# Autodesk Inventor assembly: manipulator
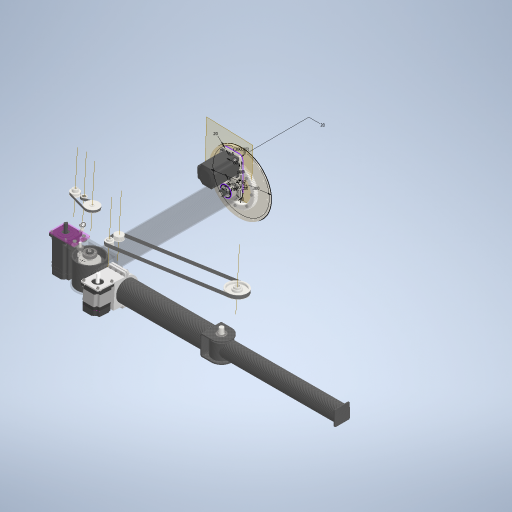
[picture p0: Inventor's stored thumbnail of the model, 512x512]
Saved by Autodesk Inventor 2023 (Build 270158000, 158)
## iProperties
Created: 2023-03-28
Part Number: manipulator
Document SubType Name: Assembly
Designer: krzys
Mass: 18520.6 g
Surface Area: 24173.7 cm^2
Volume: 7260.75 cm^3
Author: krzys
## Documents named in this file (36)
- C:\Users\krzys\Documents\GitHub\Manipulator-Inventor\Manipulator.iam
- C:\Users\krzys\Documents\GitHub\Manipulator-Inventor\podstawa.ipt
- C:\Users\krzys\Documents\GitHub\Manipulator-Inventor\podstwa_obrotowa.ipt
- C:\Users\krzys\Documents\GitHub\Manipulator-Inventor\CS-M23480_3D.ipt
- C:\Users\krzys\Documents\GitHub\Manipulator-Inventor\czlon 1 i 2.iam
- C:\Users\krzys\Documents\GitHub\Manipulator-Inventor\Manipulator\Design Accelerator\Łożysko6.iam
- C:\Users\krzys\Documents\GitHub\Manipulator-Inventor\Wał2.ipt
- C:\Users\krzys\Documents\GitHub\Manipulator-Inventor\Manipulator\Design Accelerator\Przekładnie walcowe1.iam
- C:\Users\krzys\Documents\GitHub\Manipulator-Inventor\czlon 3.ipt
- C:\Users\krzys\Documents\GitHub\Manipulator-Inventor\mocowanie silnika.ipt
- C:\Users\krzys\Documents\GitHub\Manipulator-Inventor\silniki\CS-M23485B_3D.ipt
- C:\Users\krzys\Documents\GitHub\Manipulator-Inventor\Manipulator\Design Accelerator\Przekładnie pasowe synchroniczne1.iam
- C:\Users\krzys\Documents\GitHub\Manipulator-Inventor\mocowanie_silnika_członu_3.ipt
- C:\Users\krzys\Documents\GitHub\Manipulator-Inventor\Manipulator\Design Accelerator\Przekładnie pasowe synchroniczne2.iam
- C:\Users\krzys\Documents\GitHub\Manipulator-Inventor\silniki\CS-M23445WP\CS-M23445WP_3D.iam
- C:\Users\krzys\Documents\GitHub\Manipulator-Inventor\Manipulator\Design Accelerator\Łożysko5.iam
- C:\Users\krzys\Documents\GitHub\Manipulator-Inventor\podkladka.ipt
- C:\Users\krzys\Documents\GitHub\Manipulator-Inventor\podkladka_os2.ipt
- C:\Users\krzys\Documents\Inventor\Content Center Files\R2023\pl-PL\ISO 4034(1)\ISO 4034 - M16DIN EN.ipt
- C:\Users\krzys\Documents\Inventor\Content Center Files\R2023\pl-PL\DIN 933\DIN 933 - M6  x 30.ipt
- C:\Users\krzys\Documents\Inventor\Content Center Files\R2023\pl-PL\ISO 7089\ISO 7089 - 6 - 140 HV(1).ipt
- C:\Users\krzys\Documents\Inventor\Content Center Files\R2023\pl-PL\DIN 934\DIN 934 - M6 x 1.ipt
- C:\Users\krzys\Documents\Inventor\Content Center Files\R2023\pl-PL\DIN 912\DIN 912 - M6 x 1 x 25 x 22,5.ipt
- C:\Users\krzys\Documents\Inventor\Content Center Files\R2023\pl-PL\DIN 125-1  A\DIN 125 - A 6,4.ipt
- C:\Users\krzys\Documents\Inventor\Content Center Files\R2023\pl-PL\DIN 912\DIN 912 - M6 x 1 x 20 x 17,5.ipt
- C:\Users\krzys\Documents\Inventor\Content Center Files\R2023\pl-PL\DIN 912\DIN 912 - M6 x 1 x 30 x 27,5.ipt
- C:\Users\krzys\Documents\Inventor\Content Center Files\R2023\pl-PL\DIN 933\DIN 933 - M8  x 22.ipt
- C:\Users\krzys\Documents\Inventor\Content Center Files\R2023\pl-PL\DIN 9021\DIN 9021 - 8,4.ipt
- C:\Users\krzys\Documents\Inventor\Content Center Files\R2023\pl-PL\DIN 934\DIN 934 - M8 x 1,25.ipt
- C:\Users\krzys\Documents\Inventor\Content Center Files\R2023\pl-PL\DIN 6921\DIN 6921 - M6 x 16 - A.ipt
- C:\Users\krzys\Documents\GitHub\Manipulator-Inventor\Manipulator\Design Accelerator\Łożysko7.iam
- C:\Users\krzys\Documents\GitHub\Manipulator-Inventor\Wał4.ipt
- C:\Users\krzys\Documents\Inventor\Content Center Files\R2023\pl-PL\DIN 127 - W\DIN 127 - A 6.ipt
- C:\Users\krzys\Documents\Inventor\Content Center Files\R2023\pl-PL\DIN 6921\DIN 6921 - M6 x 30 - A.ipt
- C:\Users\krzys\Documents\GitHub\Manipulator-Inventor\Manipulator\Design Accelerator\Przekładnie walcowe2.iam
- C:\Users\krzys\Documents\Inventor\Content Center Files\R2023\pl-PL\DIN 933\DIN 933 - M6  x 28.ipt
## Components (101 placed, 30 different names)
1. podstawa:1 — Wstawiające:6, Zestawiające:9, Zestawiające:80, Równoległe:7, Równoległe:8, Równoległe:9
2. podstwa_obrotowa:1 — Wstawiające:11, Wstawiające:8, Wstawiające:9, Wstawiające:25, Wstawiające:26, Wstawiające:27, Wstawiające:28, Zestawiające:52, Wstawiające:33, Wstawiające:34, Wstawiające:35, Wstawiające:36, Wstawiające:48
3. CS-M23480_3D:1 — Wstawiające:9, Wstawiające:29, Wstawiające:30, Wstawiające:31, Wstawiające:32, Zestawiające:79, Równoległe:5
4. czlon 1 i 2:1 [sub-assembly] — Wstawiające:11, Wstawiające:1, Zestawiające:6, Wstawiające:4, Wstawiające:12, Wstawiające:13, Wstawiające:14, Zestawiające:60, Zestawiające:62, Zestawiające:69, przesuwne:2
5. Łożysko:3 [sub-assembly] — Wstawiające:1, Zestawiające:72, Równoległe:4, Kątowe:1
6. Wał:1 — Zestawiające:5, Równoległe:2, Równoległe:3, Zestawiające:72, Równoległe:4, Kątowe:1
7. Przekładnie walcowe:1 [sub-assembly] — Zestawiające:5, Równoległe:2, Zestawiające:6, Równoległe:3
8. czlon 3:1 — Wstawiające:12
9. mocowanie silnika:1 — Wstawiające:38, Wstawiające:39, Wstawiające:40, Wstawiające:41, przesuwne:2
10. CS-M23485B_3D:1 — Wstawiające:40, Wstawiające:41, Wstawiające:42, Wstawiające:43, Wstawiające:44, Wstawiające:45
11. Przekładnie pasowe synchroniczne:1 [sub-assembly] — Wstawiające:46, Zestawiające:73
12. mocowanie_silnika_członu_3:1 — Wstawiające:4, Zestawiające:11, Zestawiające:12, Zestawiające:13, Zestawiające:14, Zestawiające:15, Zestawiające:16, Zestawiające:17, Zestawiające:18, Zestawiające:19, Zestawiające:20, Zestawiające:21, Zestawiające:22, Zestawiające:23, Zestawiające:24, Zestawiające:25, Zestawiające:26, Zestawiające:27, Zestawiające:28, Zestawiające:29, Zestawiające:30, Zestawiające:31, Zestawiające:32, Zestawiające:33, Zestawiające:34, Wstawiające:21, Wstawiające:22, Wstawiające:23, Wstawiające:24, Wstawiające:65
13. Przekładnie pasowe synchroniczne:2 [sub-assembly]
14. CS-M23445WP_3D:1 [sub-assembly] — Wstawiające:65, Wstawiające:66, Wstawiające:67, Wstawiające:68, Wstawiające:69
15. Łożysko:4 [sub-assembly] — Wstawiające:6, Wstawiające:48
16. Łożysko:5 [sub-assembly] — Wstawiające:8, Wstawiające:10
17. podkladka:1 — Wstawiające:10, Zestawiające:10
18. podkladka_os2:1 — Wstawiające:13, Zestawiające:8, Zestawiające:67, Zestawiające:68
19. podkladka_os2:2 — Wstawiające:14, Zestawiające:70
20. DIN EN 24034 M16:1 — Zestawiające:9, Zestawiające:10
21. DIN 933 - zastąpiona przez DIN EN 24017 M6  x 30:1 — Zestawiające:11, Zestawiające:12
22. ISO 7089 6:1 — Zestawiające:13, Zestawiające:14, Wstawiające:15
23. DIN 934 - zastąpiona przez DIN EN 24032/28673/28674 M6:1 — Wstawiające:15
24. DIN 933 - zastąpiona przez DIN EN 24017 M6  x 30:2 — Zestawiające:15, Zestawiające:16
25. ISO 7089 6:2 — Zestawiające:17, Zestawiające:18, Wstawiające:16
26. DIN 934 - zastąpiona przez DIN EN 24032/28673/28674 M6:2 — Wstawiające:16
27. DIN 933 - zastąpiona przez DIN EN 24017 M6  x 30:3 — Zestawiające:19, Zestawiające:20
28. ISO 7089 6:3 — Zestawiające:21, Zestawiające:22, Wstawiające:17
29. DIN 934 - zastąpiona przez DIN EN 24032/28673/28674 M6:3 — Wstawiające:17
30. DIN 933 - zastąpiona przez DIN EN 24017 M6  x 30:4 — Zestawiające:23, Zestawiające:24
31. ISO 7089 6:4 — Zestawiające:25, Zestawiające:26, Wstawiające:18
32. DIN 934 - zastąpiona przez DIN EN 24032/28673/28674 M6:4 — Wstawiające:18
33. DIN 933 - zastąpiona przez DIN EN 24017 M6  x 30:5 — Zestawiające:27, Zestawiające:28
34. ISO 7089 6:5 — Zestawiające:29, Zestawiające:30, Wstawiające:19
35. DIN 934 - zastąpiona przez DIN EN 24032/28673/28674 M6:5 — Wstawiające:19
36. DIN 933 - zastąpiona przez DIN EN 24017 M6  x 30:6 — Zestawiające:31, Zestawiające:32
37. ISO 7089 6:6 — Zestawiające:33, Zestawiające:34, Wstawiające:20
38. DIN 934 - zastąpiona przez DIN EN 24032/28673/28674 M6:6 — Wstawiające:20
39. DIN 125-1 A A 6,4:1 — Wstawiające:21, Wstawiające:73
40. DIN 125-1 A A 6,4:2 — Wstawiające:22, Wstawiające:70
41. DIN 125-1 A A 6,4:3 — Wstawiające:23, Wstawiające:72
42. DIN 125-1 A A 6,4:4 — Wstawiające:24, Wstawiające:71
43. DIN 912 - zastąpiona przez DIN EN ISO 4762 M6 x 20:1 — Wstawiające:25
44. DIN 912 - zastąpiona przez DIN EN ISO 4762 M6 x 20:2 — Wstawiające:26
45. DIN 912 - zastąpiona przez DIN EN ISO 4762 M6 x 20:3 — Wstawiające:27
46. DIN 912 - zastąpiona przez DIN EN ISO 4762 M6 x 20:4 — Wstawiające:28
47. DIN 912 - zastąpiona przez DIN EN ISO 4762 M6 x 30:1 — Wstawiające:29, Zestawiające:51, Zestawiające:53
48. DIN 912 - zastąpiona przez DIN EN ISO 4762 M6 x 30:2 — Wstawiające:30, Zestawiające:55
49. DIN 912 - zastąpiona przez DIN EN ISO 4762 M6 x 30:3 — Wstawiające:31, Zestawiające:57
50. DIN 912 - zastąpiona przez DIN EN ISO 4762 M6 x 30:4 — Wstawiające:32
51. DIN 125-1 A A 6,4:5 — Zestawiające:51, Zestawiające:52, Zestawiające:54
52. DIN 125-1 A A 6,4:6 — Wstawiające:33, Zestawiające:56
53. DIN 125-1 A A 6,4:7 — Wstawiające:34, Wstawiające:37
54. DIN 125-1 A A 6,4:8 — Wstawiające:35
55. DIN 125-1 A A 6,4:9 — Wstawiające:36, Zestawiające:58
56. DIN 934 - zastąpiona przez DIN EN 24032/28673/28674 M6:11 — Zestawiające:53, Zestawiające:54
57. DIN 934 - zastąpiona przez DIN EN 24032/28673/28674 M6:12 — Zestawiające:55, Zestawiające:56
58. DIN 934 - zastąpiona przez DIN EN 24032/28673/28674 M6:13 — Wstawiające:37
59. DIN 934 - zastąpiona przez DIN EN 24032/28673/28674 M6:14 — Zestawiające:57, Zestawiające:58
60. DIN 933 - zastąpiona przez DIN EN 24017 M8  x 22:1 — Wstawiające:38, Zestawiające:59, Zestawiające:63
61. DIN 933 - zastąpiona przez DIN EN 24017 M8  x 22:2 — Wstawiające:39, Zestawiające:61, Zestawiające:65
62. DIN 9021 8,4:1 — Zestawiające:59, Zestawiające:60, Zestawiające:64
63. DIN 9021 8,4:2 — Zestawiające:61, Zestawiające:62, Zestawiające:66
64. DIN 934 - zastąpiona przez DIN EN 24032/28673/28674 M8:1 — Zestawiające:63, Zestawiające:64
65. DIN 934 - zastąpiona przez DIN EN 24032/28673/28674 M8:2 — Zestawiające:65, Zestawiające:66
66. DIN 912 - zastąpiona przez DIN EN ISO 4762 M6 x 20:5 — Wstawiające:42
67. DIN 912 - zastąpiona przez DIN EN ISO 4762 M6 x 20:6 — Wstawiające:43
68. DIN 912 - zastąpiona przez DIN EN ISO 4762 M6 x 20:7 — Wstawiające:44
69. DIN 912 - zastąpiona przez DIN EN ISO 4762 M6 x 20:8 — Wstawiające:45
70. DIN 6921 M6 x 16:1 — Zestawiające:67, Zestawiające:68
71. DIN 6921 M6 x 16:2 — Zestawiające:69, Zestawiające:70
72. Łożysko:6 [sub-assembly] — Wstawiające:46
73. Wał:1 — Zestawiające:73, Zestawiające:75, Zestawiające:76, Zestawiające:77
74. DIN 9021 8,4:3 — Zestawiające:75, Zestawiające:76, Zestawiające:78
75. DIN 127 - wycofana A 6:1 — Zestawiające:77, Zestawiające:78, Wstawiające:47
76. DIN 6921 M6 x 30:1 — Wstawiające:47
77. Przekładnie walcowe:2 [sub-assembly] — Zestawiające:79, Równoległe:5, Zestawiające:80, Równoległe:6, Wstawiające:49, Wstawiające:50, Wstawiające:51, Wstawiające:52, Wstawiające:53, Wstawiające:54, Wstawiające:55, Wstawiające:56
78. DIN 125-1 A A 6,4:10 — Wstawiające:49, Wstawiające:58
79. DIN 125-1 A A 6,4:11 — Wstawiające:50, Wstawiające:64
80. DIN 125-1 A A 6,4:12 — Wstawiające:51, Wstawiające:57
81. DIN 125-1 A A 6,4:13 — Wstawiające:52, Wstawiające:59
82. DIN 125-1 A A 6,4:14 — Wstawiające:53, Wstawiające:63
83. DIN 125-1 A A 6,4:15 — Wstawiające:54, Wstawiające:60
84. DIN 125-1 A A 6,4:16 — Wstawiające:55, Wstawiające:61
85. DIN 125-1 A A 6,4:17 — Wstawiające:56, Wstawiające:62
86. DIN 933 - zastąpiona przez DIN EN 24017 M6  x 28:1 — Wstawiające:57
87. DIN 933 - zastąpiona przez DIN EN 24017 M6  x 28:2 — Wstawiające:58
88. DIN 933 - zastąpiona przez DIN EN 24017 M6  x 28:3 — Wstawiające:59
89. DIN 933 - zastąpiona przez DIN EN 24017 M6  x 28:4 — Wstawiające:60
90. DIN 933 - zastąpiona przez DIN EN 24017 M6  x 28:5 — Wstawiające:61
91. DIN 933 - zastąpiona przez DIN EN 24017 M6  x 28:6 — Wstawiające:62
92. DIN 933 - zastąpiona przez DIN EN 24017 M6  x 28:7 — Wstawiające:63
93. DIN 933 - zastąpiona przez DIN EN 24017 M6  x 28:8 — Wstawiające:64
94. DIN 912 - zastąpiona przez DIN EN ISO 4762 M6 x 25:1 — Wstawiające:66
95. DIN 912 - zastąpiona przez DIN EN ISO 4762 M6 x 25:2 — Wstawiające:67
96. DIN 912 - zastąpiona przez DIN EN ISO 4762 M6 x 25:3 — Wstawiające:68
97. DIN 912 - zastąpiona przez DIN EN ISO 4762 M6 x 25:4 — Wstawiające:69
98. DIN 934 - zastąpiona przez DIN EN 24032/28673/28674 M6:15 — Wstawiające:70
99. DIN 934 - zastąpiona przez DIN EN 24032/28673/28674 M6:16 — Wstawiające:71
100. DIN 934 - zastąpiona przez DIN EN 24032/28673/28674 M6:17 — Wstawiające:72
101. DIN 934 - zastąpiona przez DIN EN 24032/28673/28674 M6:18 — Wstawiające:73
## Relationships (136: Insert 69, Mate 57, Flush 8, TranslationJoint 1, Angle 1)
- Wstawiające:11 [Insert]: podstwa_obrotowa:1 ↔ czlon 1 i 2:1
- Wstawiające:1 [Insert]: czlon 1 i 2:1 ↔ Łożysko:3
- Zestawiające:5 [Mate]: Wał:1 ↔ Przekładnie walcowe:1
- Równoległe:2 [Flush]: Wał:1 ↔ Przekładnie walcowe:1
- Zestawiające:6 [Mate]: czlon 1 i 2:1 ↔ Przekładnie walcowe:1
- Równoległe:3 [Flush]: Wał:1 ↔ Przekładnie walcowe:1
- Wstawiające:4 [Insert] (-500 mm): czlon 1 i 2:1 ↔ mocowanie_silnika_członu_3:1
- Wstawiające:6 [Insert] (-1 mm): podstawa:1 ↔ Łożysko:4
- Wstawiające:8 [Insert] (1 mm): podstwa_obrotowa:1 ↔ Łożysko:5
- Wstawiające:9 [Insert]: podstwa_obrotowa:1 ↔ CS-M23480_3D:1
- Wstawiające:10 [Insert]: Łożysko:5 ↔ podkladka:1
- Wstawiające:12 [Insert] (40.5 mm): czlon 1 i 2:1 ↔ czlon 3:1
- Wstawiające:13 [Insert]: czlon 1 i 2:1 ↔ podkladka_os2:1
- Wstawiające:14 [Insert]: czlon 1 i 2:1 ↔ podkladka_os2:2
- Zestawiające:8 [Mate]: podkladka_os2:1
- Zestawiające:9 [Mate]: podstawa:1 ↔ DIN EN 24034 M16:1
- Zestawiające:10 [Mate]: podkladka:1 ↔ DIN EN 24034 M16:1
- Zestawiające:11 [Mate]: mocowanie_silnika_członu_3:1 ↔ DIN 933 - zastąpiona przez DIN EN 24017 M6  x 30:1
- Zestawiające:12 [Mate]: mocowanie_silnika_członu_3:1 ↔ DIN 933 - zastąpiona przez DIN EN 24017 M6  x 30:1
- Zestawiające:13 [Mate]: mocowanie_silnika_członu_3:1 ↔ ISO 7089 6:1
- Zestawiające:14 [Mate]: mocowanie_silnika_członu_3:1 ↔ ISO 7089 6:1
- Wstawiające:15 [Insert]: ISO 7089 6:1 ↔ DIN 934 - zastąpiona przez DIN EN 24032/28673/28674 M6:1
- Zestawiające:15 [Mate]: mocowanie_silnika_członu_3:1 ↔ DIN 933 - zastąpiona przez DIN EN 24017 M6  x 30:2
- Zestawiające:16 [Mate]: mocowanie_silnika_członu_3:1 ↔ DIN 933 - zastąpiona przez DIN EN 24017 M6  x 30:2
- Zestawiające:17 [Mate]: mocowanie_silnika_członu_3:1 ↔ ISO 7089 6:2
- Zestawiające:18 [Mate]: mocowanie_silnika_członu_3:1 ↔ ISO 7089 6:2
- Wstawiające:16 [Insert]: ISO 7089 6:2 ↔ DIN 934 - zastąpiona przez DIN EN 24032/28673/28674 M6:2
- Zestawiające:19 [Mate]: mocowanie_silnika_członu_3:1 ↔ DIN 933 - zastąpiona przez DIN EN 24017 M6  x 30:3
- Zestawiające:20 [Mate]: mocowanie_silnika_członu_3:1 ↔ DIN 933 - zastąpiona przez DIN EN 24017 M6  x 30:3
- Zestawiające:21 [Mate]: mocowanie_silnika_członu_3:1 ↔ ISO 7089 6:3
- Zestawiające:22 [Mate]: mocowanie_silnika_członu_3:1 ↔ ISO 7089 6:3
- Wstawiające:17 [Insert]: ISO 7089 6:3 ↔ DIN 934 - zastąpiona przez DIN EN 24032/28673/28674 M6:3
- Zestawiające:23 [Mate]: mocowanie_silnika_członu_3:1 ↔ DIN 933 - zastąpiona przez DIN EN 24017 M6  x 30:4
- Zestawiające:24 [Mate]: mocowanie_silnika_członu_3:1 ↔ DIN 933 - zastąpiona przez DIN EN 24017 M6  x 30:4
- Zestawiające:25 [Mate]: mocowanie_silnika_członu_3:1 ↔ ISO 7089 6:4
- Zestawiające:26 [Mate]: mocowanie_silnika_członu_3:1 ↔ ISO 7089 6:4
- Wstawiające:18 [Insert]: ISO 7089 6:4 ↔ DIN 934 - zastąpiona przez DIN EN 24032/28673/28674 M6:4
- Zestawiające:27 [Mate]: mocowanie_silnika_członu_3:1 ↔ DIN 933 - zastąpiona przez DIN EN 24017 M6  x 30:5
- Zestawiające:28 [Mate]: mocowanie_silnika_członu_3:1 ↔ DIN 933 - zastąpiona przez DIN EN 24017 M6  x 30:5
- Zestawiające:29 [Mate]: mocowanie_silnika_członu_3:1 ↔ ISO 7089 6:5
- Zestawiające:30 [Mate]: mocowanie_silnika_członu_3:1 ↔ ISO 7089 6:5
- Wstawiające:19 [Insert]: ISO 7089 6:5 ↔ DIN 934 - zastąpiona przez DIN EN 24032/28673/28674 M6:5
- Zestawiające:31 [Mate]: mocowanie_silnika_członu_3:1 ↔ DIN 933 - zastąpiona przez DIN EN 24017 M6  x 30:6
- Zestawiające:32 [Mate]: mocowanie_silnika_członu_3:1 ↔ DIN 933 - zastąpiona przez DIN EN 24017 M6  x 30:6
- Zestawiające:33 [Mate]: mocowanie_silnika_członu_3:1 ↔ ISO 7089 6:6
- Zestawiające:34 [Mate]: mocowanie_silnika_członu_3:1 ↔ ISO 7089 6:6
- Wstawiające:20 [Insert]: ISO 7089 6:6 ↔ DIN 934 - zastąpiona przez DIN EN 24032/28673/28674 M6:6
- Wstawiające:21 [Insert]: mocowanie_silnika_członu_3:1 ↔ DIN 125-1 A A 6,4:1
- Wstawiające:22 [Insert]: mocowanie_silnika_członu_3:1 ↔ DIN 125-1 A A 6,4:2
- Wstawiające:23 [Insert]: mocowanie_silnika_członu_3:1 ↔ DIN 125-1 A A 6,4:3
- Wstawiające:24 [Insert]: mocowanie_silnika_członu_3:1 ↔ DIN 125-1 A A 6,4:4
- Wstawiające:25 [Insert]: podstwa_obrotowa:1 ↔ DIN 912 - zastąpiona przez DIN EN ISO 4762 M6 x 20:1
- Wstawiające:26 [Insert]: podstwa_obrotowa:1 ↔ DIN 912 - zastąpiona przez DIN EN ISO 4762 M6 x 20:2
- Wstawiające:27 [Insert]: podstwa_obrotowa:1 ↔ DIN 912 - zastąpiona przez DIN EN ISO 4762 M6 x 20:3
- Wstawiające:28 [Insert]: podstwa_obrotowa:1 ↔ DIN 912 - zastąpiona przez DIN EN ISO 4762 M6 x 20:4
- Wstawiające:29 [Insert]: CS-M23480_3D:1 ↔ DIN 912 - zastąpiona przez DIN EN ISO 4762 M6 x 30:1
- Wstawiające:30 [Insert]: CS-M23480_3D:1 ↔ DIN 912 - zastąpiona przez DIN EN ISO 4762 M6 x 30:2
- Wstawiające:31 [Insert]: CS-M23480_3D:1 ↔ DIN 912 - zastąpiona przez DIN EN ISO 4762 M6 x 30:3
- Wstawiające:32 [Insert]: CS-M23480_3D:1 ↔ DIN 912 - zastąpiona przez DIN EN ISO 4762 M6 x 30:4
- Zestawiające:51 [Mate]: DIN 912 - zastąpiona przez DIN EN ISO 4762 M6 x 30:1 ↔ DIN 125-1 A A 6,4:5
- Zestawiające:52 [Mate]: podstwa_obrotowa:1 ↔ DIN 125-1 A A 6,4:5
- Wstawiające:33 [Insert]: podstwa_obrotowa:1 ↔ DIN 125-1 A A 6,4:6
- Wstawiające:34 [Insert]: podstwa_obrotowa:1 ↔ DIN 125-1 A A 6,4:7
- Wstawiające:35 [Insert]: podstwa_obrotowa:1 ↔ DIN 125-1 A A 6,4:8
- Wstawiające:36 [Insert]: podstwa_obrotowa:1 ↔ DIN 125-1 A A 6,4:9
- Zestawiające:53 [Mate]: DIN 912 - zastąpiona przez DIN EN ISO 4762 M6 x 30:1 ↔ DIN 934 - zastąpiona przez DIN EN 24032/28673/28674 M6:11
- Zestawiające:54 [Mate]: DIN 125-1 A A 6,4:5 ↔ DIN 934 - zastąpiona przez DIN EN 24032/28673/28674 M6:11
- Zestawiające:55 [Mate]: DIN 912 - zastąpiona przez DIN EN ISO 4762 M6 x 30:2 ↔ DIN 934 - zastąpiona przez DIN EN 24032/28673/28674 M6:12
- Zestawiające:56 [Mate]: DIN 125-1 A A 6,4:6 ↔ DIN 934 - zastąpiona przez DIN EN 24032/28673/28674 M6:12
- Wstawiające:37 [Insert]: DIN 125-1 A A 6,4:7 ↔ DIN 934 - zastąpiona przez DIN EN 24032/28673/28674 M6:13
- Zestawiające:57 [Mate]: DIN 912 - zastąpiona przez DIN EN ISO 4762 M6 x 30:3 ↔ DIN 934 - zastąpiona przez DIN EN 24032/28673/28674 M6:14
- Zestawiające:58 [Mate]: DIN 125-1 A A 6,4:9 ↔ DIN 934 - zastąpiona przez DIN EN 24032/28673/28674 M6:14
- Wstawiające:38 [Insert]: mocowanie silnika:1 ↔ DIN 933 - zastąpiona przez DIN EN 24017 M8  x 22:1
- Wstawiające:39 [Insert]: mocowanie silnika:1 ↔ DIN 933 - zastąpiona przez DIN EN 24017 M8  x 22:2
- Zestawiające:59 [Mate]: DIN 933 - zastąpiona przez DIN EN 24017 M8  x 22:1 ↔ DIN 9021 8,4:1
- Zestawiające:60 [Mate]: czlon 1 i 2:1 ↔ DIN 9021 8,4:1
- Zestawiające:61 [Mate]: DIN 933 - zastąpiona przez DIN EN 24017 M8  x 22:2 ↔ DIN 9021 8,4:2
- Zestawiające:62 [Mate]: czlon 1 i 2:1 ↔ DIN 9021 8,4:2
- Zestawiające:63 [Mate]: DIN 933 - zastąpiona przez DIN EN 24017 M8  x 22:1 ↔ DIN 934 - zastąpiona przez DIN EN 24032/28673/28674 M8:1
- Zestawiające:64 [Mate]: DIN 9021 8,4:1 ↔ DIN 934 - zastąpiona przez DIN EN 24032/28673/28674 M8:1
- Zestawiające:65 [Mate]: DIN 933 - zastąpiona przez DIN EN 24017 M8  x 22:2 ↔ DIN 934 - zastąpiona przez DIN EN 24032/28673/28674 M8:2
- Zestawiające:66 [Mate]: DIN 9021 8,4:2 ↔ DIN 934 - zastąpiona przez DIN EN 24032/28673/28674 M8:2
- Wstawiające:40 [Insert] (-0.5 mm): mocowanie silnika:1 ↔ CS-M23485B_3D:1
- Wstawiające:41 [Insert] (0.5 mm): mocowanie silnika:1 ↔ CS-M23485B_3D:1
- Wstawiające:42 [Insert]: CS-M23485B_3D:1 ↔ DIN 912 - zastąpiona przez DIN EN ISO 4762 M6 x 20:5
- Wstawiające:43 [Insert]: CS-M23485B_3D:1 ↔ DIN 912 - zastąpiona przez DIN EN ISO 4762 M6 x 20:6
- Wstawiające:44 [Insert]: CS-M23485B_3D:1 ↔ DIN 912 - zastąpiona przez DIN EN ISO 4762 M6 x 20:7
- Wstawiające:45 [Insert]: CS-M23485B_3D:1 ↔ DIN 912 - zastąpiona przez DIN EN ISO 4762 M6 x 20:8
- Zestawiające:67 [Mate]: podkladka_os2:1 ↔ DIN 6921 M6 x 16:1
- Zestawiające:68 [Mate]: podkladka_os2:1 ↔ DIN 6921 M6 x 16:1
- Zestawiające:69 [Mate]: czlon 1 i 2:1 ↔ DIN 6921 M6 x 16:2
- Zestawiające:70 [Mate]: podkladka_os2:2 ↔ DIN 6921 M6 x 16:2
- przesuwne:2 [TranslationJoint]: czlon 1 i 2:1 ↔ mocowanie silnika:1
- Zestawiające:72 [Mate]: Łożysko:3 ↔ Wał:1
- Równoległe:4 [Flush] (-20 mm): Łożysko:3 ↔ Wał:1
- Kątowe:1 [Angle] (0 deg): Łożysko:3 ↔ Wał:1
- Wstawiające:46 [Insert]: Przekładnie pasowe synchroniczne:1 ↔ Łożysko:6
- Zestawiające:73 [Mate]: Przekładnie pasowe synchroniczne:1 ↔ Wał:1
- Zestawiające:75 [Mate]: Wał:1 ↔ DIN 9021 8,4:3
- Zestawiające:76 [Mate]: Wał:1 ↔ DIN 9021 8,4:3
- Zestawiające:77 [Mate]: Wał:1 ↔ DIN 127 - wycofana A 6:1
- Zestawiające:78 [Mate]: DIN 9021 8,4:3 ↔ DIN 127 - wycofana A 6:1
- Wstawiające:47 [Insert]: DIN 127 - wycofana A 6:1 ↔ DIN 6921 M6 x 30:1
- Wstawiające:48 [Insert]: podstwa_obrotowa:1 ↔ Łożysko:4
- Zestawiające:79 [Mate]: CS-M23480_3D:1 ↔ Przekładnie walcowe:2
- Równoległe:5 [Flush]: CS-M23480_3D:1 ↔ Przekładnie walcowe:2
- Zestawiające:80 [Mate]: podstawa:1 ↔ Przekładnie walcowe:2
- Równoległe:6 [Flush]: Przekładnie walcowe:2
- Równoległe:7 [Flush]: podstawa:1
- Równoległe:8 [Flush]: podstawa:1
- Równoległe:9 [Flush]: podstawa:1
- Wstawiające:49 [Insert]: Przekładnie walcowe:2 ↔ DIN 125-1 A A 6,4:10
- Wstawiające:50 [Insert]: Przekładnie walcowe:2 ↔ DIN 125-1 A A 6,4:11
- Wstawiające:51 [Insert]: Przekładnie walcowe:2 ↔ DIN 125-1 A A 6,4:12
- Wstawiające:52 [Insert]: Przekładnie walcowe:2 ↔ DIN 125-1 A A 6,4:13
- Wstawiające:53 [Insert]: Przekładnie walcowe:2 ↔ DIN 125-1 A A 6,4:14
- Wstawiające:54 [Insert]: Przekładnie walcowe:2 ↔ DIN 125-1 A A 6,4:15
- Wstawiające:55 [Insert]: Przekładnie walcowe:2 ↔ DIN 125-1 A A 6,4:16
- Wstawiające:56 [Insert]: Przekładnie walcowe:2 ↔ DIN 125-1 A A 6,4:17
- Wstawiające:57 [Insert]: DIN 125-1 A A 6,4:12 ↔ DIN 933 - zastąpiona przez DIN EN 24017 M6  x 28:1
- Wstawiające:58 [Insert]: DIN 125-1 A A 6,4:10 ↔ DIN 933 - zastąpiona przez DIN EN 24017 M6  x 28:2
- Wstawiające:59 [Insert]: DIN 125-1 A A 6,4:13 ↔ DIN 933 - zastąpiona przez DIN EN 24017 M6  x 28:3
- Wstawiające:60 [Insert]: DIN 125-1 A A 6,4:15 ↔ DIN 933 - zastąpiona przez DIN EN 24017 M6  x 28:4
- Wstawiające:61 [Insert]: DIN 125-1 A A 6,4:16 ↔ DIN 933 - zastąpiona przez DIN EN 24017 M6  x 28:5
- Wstawiające:62 [Insert]: DIN 125-1 A A 6,4:17 ↔ DIN 933 - zastąpiona przez DIN EN 24017 M6  x 28:6
- Wstawiające:63 [Insert]: DIN 125-1 A A 6,4:14 ↔ DIN 933 - zastąpiona przez DIN EN 24017 M6  x 28:7
- Wstawiające:64 [Insert]: DIN 125-1 A A 6,4:11 ↔ DIN 933 - zastąpiona przez DIN EN 24017 M6  x 28:8
- Wstawiające:65 [Insert]: mocowanie_silnika_członu_3:1 ↔ CS-M23445WP_3D:1
- Wstawiające:66 [Insert]: CS-M23445WP_3D:1 ↔ DIN 912 - zastąpiona przez DIN EN ISO 4762 M6 x 25:1
- Wstawiające:67 [Insert]: CS-M23445WP_3D:1 ↔ DIN 912 - zastąpiona przez DIN EN ISO 4762 M6 x 25:2
- Wstawiające:68 [Insert]: CS-M23445WP_3D:1 ↔ DIN 912 - zastąpiona przez DIN EN ISO 4762 M6 x 25:3
- Wstawiające:69 [Insert]: CS-M23445WP_3D:1 ↔ DIN 912 - zastąpiona przez DIN EN ISO 4762 M6 x 25:4
- Wstawiające:70 [Insert]: DIN 125-1 A A 6,4:2 ↔ DIN 934 - zastąpiona przez DIN EN 24032/28673/28674 M6:15
- Wstawiające:71 [Insert]: DIN 125-1 A A 6,4:4 ↔ DIN 934 - zastąpiona przez DIN EN 24032/28673/28674 M6:16
- Wstawiające:72 [Insert]: DIN 125-1 A A 6,4:3 ↔ DIN 934 - zastąpiona przez DIN EN 24032/28673/28674 M6:17
- Wstawiające:73 [Insert]: DIN 125-1 A A 6,4:1 ↔ DIN 934 - zastąpiona przez DIN EN 24032/28673/28674 M6:18
